# Autodesk Inventor assembly: Assembly_Cube_Z_Focus_Drylin_NEMA_v3
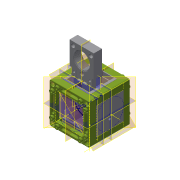
[picture p0: Inventor's stored thumbnail of the model, 180x180]
Saved by Autodesk Inventor 2022 (Build 260153000, 153)
## iProperties
Created: 2021-04-25
Part Number: Assembly_Cube_Z_Focus_Drylin_NEMA_v3
Document SubType Name: Assembly
Designer: diederichbenedict
Author: diederichbenedict
## Documents named in this file (8)
- C:\Users\PrakashLab\Documents\UC2-INVENTOR-Git\uc2_v3\Assembly_Cube_Z_Focus_Drylin_manual_v3.iam
- C:\Users\PrakashLab\Documents\UC2-Zstage\INVENTOR\Assembly_Cube_empty_IM_v3.iam
- C:\Users\PrakashLab\Documents\UC2-INVENTOR-Git\uc2_v3\10_Base_puzzle_v3.ipt
- C:\Users\PrakashLab\Documents\UC2-INVENTOR-Git\uc2_v3\00_rod_6mm.ipt
- C:\Users\PrakashLab\Documents\UC2-INVENTOR-Git\uc2_v3\30_Cube_Z_Focus_Drylin_manual_base_v3.ipt
- C:\Users\PrakashLab\Documents\UC2-INVENTOR-Git\uc2_v3\30_Cube_Z_Focus_Drylin_manual_slide.ipt
- C:\Users\PrakashLab\Documents\UC2-INVENTOR-Git\uc2_v3\30_Cube_Z_Focus_MGN12_manual_gear_v3.ipt
- C:\Users\PrakashLab\Documents\UC2-INVENTOR-Git\uc2_v3\30_Cube_Z_Focus_MGN_NEMA_adapter_RMS.ipt
## Components (11 placed, 7 different names)
1. 30_Cube_Z_Focus_MGN_NEMA_adapter_RMS:1 — Insert:8, Angle:1
2. 00_rod_6mm:2 — Mate:15
3. 00_rod_6mm:3
4. 30_Cube_Z_Focus_Drylin_manual_base_v3:1 — Flush:15, Mate:13, Mate:14, Insert:7, Mate:16, Mate:17, Mate:18, Mate:19
5. 30_Cube_Z_Focus_MGN12_manual_gear_v3:1 — Insert:7
6. 30_Cube_Z_Focus_Drylin_manual_slide:1 — Mate:15, Mate:16, Insert:8, Angle:1
7. Assembly_Cube_empty_IM_v3:4 [sub-assembly] — Mate:17, Mate:18, Mate:19
8. 10_Base_puzzle_v3:1 — Insert:6
9. 10_Base_puzzle_v3:2
10. Assembly_Cube_empty_IM_v3:1 [sub-assembly] — Insert:6, Flush:15, Mate:13, Mate:14
11. Assembly_Cube_empty_IM_v3:3 [sub-assembly]
## Component patterns: (2 elements, first: 10_Base_puzzle_v3:1), (2 elements, first: Assembly_Cube_empty_IM_v3:1)
## Relationships (12: Mate 7, Insert 3, Flush 1, Angle 1)
- Insert:6: 10_Base_puzzle_v3:1 ↔ Assembly_Cube_empty_IM_v3:1
- Flush:15: 30_Cube_Z_Focus_Drylin_manual_base_v3:1 ↔ Assembly_Cube_empty_IM_v3:1
- Mate:13: 30_Cube_Z_Focus_Drylin_manual_base_v3:1 ↔ Assembly_Cube_empty_IM_v3:1
- Mate:14: 30_Cube_Z_Focus_Drylin_manual_base_v3:1 ↔ Assembly_Cube_empty_IM_v3:1
- Insert:7: 30_Cube_Z_Focus_Drylin_manual_base_v3:1 ↔ 30_Cube_Z_Focus_MGN12_manual_gear_v3:1
- Mate:15: 00_rod_6mm:2 ↔ 30_Cube_Z_Focus_Drylin_manual_slide:1
- Mate:16 (-25 mm): 30_Cube_Z_Focus_Drylin_manual_base_v3:1 ↔ 30_Cube_Z_Focus_Drylin_manual_slide:1
- Insert:8: 30_Cube_Z_Focus_MGN_NEMA_adapter_RMS:1 ↔ 30_Cube_Z_Focus_Drylin_manual_slide:1
- Angle:1 (0 deg): 30_Cube_Z_Focus_MGN_NEMA_adapter_RMS:1 ↔ 30_Cube_Z_Focus_Drylin_manual_slide:1
- Mate:17: 30_Cube_Z_Focus_Drylin_manual_base_v3:1 ↔ Assembly_Cube_empty_IM_v3:4
- Mate:18: 30_Cube_Z_Focus_Drylin_manual_base_v3:1 ↔ Assembly_Cube_empty_IM_v3:4
- Mate:19: 30_Cube_Z_Focus_Drylin_manual_base_v3:1 ↔ Assembly_Cube_empty_IM_v3:4
